# Autodesk Inventor assembly: 1.625 od Flex with ersa
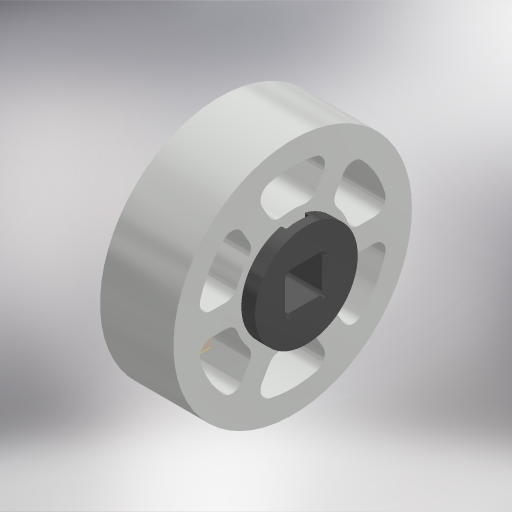
[picture p0: Inventor's stored thumbnail of the model, 512x512]
Saved by Autodesk Inventor 2023 (Build 270158000, 158)
## iProperties
Created: 2022-12-12
Part Number: 1.625 od Flex with ersa
Document SubType Name: Assembly
Designer: aaron
Author: aaron
## Documents named in this file (3)
- C:\Users\aaron\Documents\Inventor\Spin Up\library\Motion\Flex Wheels\1.625 od Flex with ersa.iam
- C:\Users\aaron\Documents\Inventor\Spin Up\library\Motion\Flex Wheels\1.625 OD flex.ipt
- C:\Users\aaron\Documents\Inventor\Spin Up\library\Motion\Flex Wheels\small versa.ipt
## Components (3 placed, 2 different names)
1. 1.625 OD flex:1 — Mate:1, Mate:2, Mate:3, Mate:4
2. small versa:1 — Mate:1, Mate:2, Flush:1, Symmetry:1
3. small versa:2 — Mate:3, Mate:4, Flush:1, Symmetry:1
## Relationships (6: Mate 4, Flush 1, Symmetry 1)
- Mate:1: 1.625 OD flex:1 ↔ small versa:1
- Mate:2: 1.625 OD flex:1 ↔ small versa:1
- Mate:3: 1.625 OD flex:1 ↔ small versa:2
- Mate:4: 1.625 OD flex:1 ↔ small versa:2
- Flush:1: small versa:1 ↔ small versa:2
- Symmetry:1: small versa:1 ↔ small versa:2
